# Autodesk Inventor assembly: Custoboard
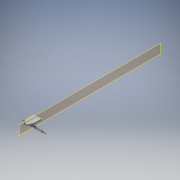
[picture p0: Inventor's stored thumbnail of the model, 180x180]
Saved by Autodesk Inventor 2018 (Build 220112000, 112)
## iProperties
Created: 2017-09-12
Part Number: Custoboard
Document SubType Name: Assembly
Designer: Rus
Author: Rus
## Documents named in this file (11)
- E:\Libraries\Documents\3D Models\Electric Longboard\Custoboard.iam
- E:\Libraries\Documents\3D Models\Electric Longboard\Trucks\50_CAL\10cal_hanger.ipt
- E:\Libraries\Documents\3D Models\Electric Longboard\Trucks\50_CAL\50cal_baseplate.ipt
- E:\Libraries\Documents\3D Models\Electric Longboard\Trucks\50_CAL\BS_bushing.ipt
- E:\Libraries\Documents\3D Models\Electric Longboard\Trucks\50_CAL\RS_washer.ipt
- E:\Libraries\Documents\3D Models\Electric Longboard\Trucks\50_CAL\RS_bushing.ipt
- E:\Libraries\Documents\3D Models\Electric Longboard\Trucks\50_CAL\Pivot_cup.ipt
- E:\Libraries\Documents\3D Models\Electric Longboard\Trucks\50_CAL\kingpin-nut.ipt
- E:\Libraries\Documents\3D Models\Electric Longboard\Trucks\50_CAL\kingpin.ipt
- E:\Libraries\Documents\3D Models\Electric Longboard\Trucks\50_CAL\BS_washer.ipt
- E:\Libraries\Documents\3D Models\Electric Longboard\Boards\TempAllBoard.ipt
## Components (10 placed, 10 different names)
1. TempAllBoard:1 — Angle:1, Insert:17, Mate:11, Angle:7
2. 10cal_hanger:1 — Rotational:1
3. 50cal_baseplate:1 — Angle:1, Insert:9, Angle:2, Insert:10, Angle:3, Insert:17, Angle:9, Angle:11, Mate:15, Insert:18
4. BS_bushing:2 — Insert:11
5. RS_washer:1 — Insert:13, Insert:14
6. RS_bushing:1 — Insert:14
7. kingpin-nut:1 — Insert:12, Insert:13, Angle:3
8. kingpin:1 — Insert:9, Angle:2, Insert:12
9. BS_washer:3 — Insert:10, Insert:11
10. Pivot_cup:1 — Mate:13, Mate:14, Angle:10, Mate:15, Insert:18, Rotational:1
## Relationships (21: Angle 8, Insert 8, Mate 4, RevoluteJoint 1)
- Angle:1 (0 deg): TempAllBoard:1 ↔ 50cal_baseplate:1
- Insert:9: 50cal_baseplate:1 ↔ kingpin:1
- Angle:2 (60 deg): 50cal_baseplate:1 ↔ kingpin:1
- Insert:10: 50cal_baseplate:1 ↔ BS_washer:3
- Insert:11: BS_bushing:2 ↔ BS_washer:3
- Insert:12: kingpin-nut:1 ↔ kingpin:1
- Insert:13: RS_washer:1 ↔ kingpin-nut:1
- Insert:14: RS_washer:1 ↔ RS_bushing:1
- Angle:3 (0 deg): 50cal_baseplate:1 ↔ kingpin-nut:1
- Insert:17: TempAllBoard:1 ↔ 50cal_baseplate:1
- Mate:11: TempAllBoard:1
- Angle:7 (0 deg): TempAllBoard:1
- Mate:13: Pivot_cup:1
- Angle:8 (0 deg)
- Angle:9 (90 deg): 50cal_baseplate:1
- Mate:14: Pivot_cup:1
- Angle:10 (0 deg): Pivot_cup:1
- Angle:11 (0 deg): 50cal_baseplate:1
- Mate:15: 50cal_baseplate:1 ↔ Pivot_cup:1
- Insert:18: 50cal_baseplate:1 ↔ Pivot_cup:1
- Rotational:1 [RevoluteJoint]: 10cal_hanger:1 ↔ Pivot_cup:1
